# Autodesk Inventor assembly: PlattaAssembly
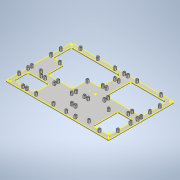
[picture p0: Inventor's stored thumbnail of the model, 180x180]
Saved by Autodesk Inventor 2021 (Build 250183000, 183)
## iProperties
Created: 2020-02-26
Part Number: PlattaAssembly
Document SubType Name: Assembly
Designer: lgnds
Author: lgnds
## Documents named in this file (3)
- C:\Users\Viktor\Documents\GitHub\WaveRunner-CCU\CCU_Assembly\hw\CAD\PlattaAssembly.iam
- C:\Users\Viktor\Documents\GitHub\WaveRunner-CCU\CCU_Assembly\hw\CAD\Platta.ipt
- C:\Users\Viktor\Documents\GitHub\WaveRunner-CCU\CCU_Assembly\hw\CAD\Other\Spacer7mm_m3_970070321.ipt
## Components (49 placed, 2 different names)
1. Platta:1 — Rigid:1, Rigid:2, Rigid:3, Rigid:4, Rigid:5, Rigid:6, Rigid:7, Rigid:8, Rigid:9, Rigid:10, Rigid:11, Rigid:12, Rigid:13, Rigid:14, Rigid:15, Rigid:16, Rigid:17, Rigid:18, Rigid:19, Rigid:20, Rigid:21, Rigid:22, Rigid:23, Rigid:24, Rigid:25, Rigid:26, Rigid:27, Rigid:28, Rigid:29, Rigid:30, Rigid:31, Rigid:32, Rigid:33, Rigid:34, Rigid:35, Rigid:36, Rigid:37, Rigid:38, Rigid:39, Rigid:40, Rigid:41, Rigid:42, Rigid:43, Rigid:44, Rigid:45, Rigid:46, Rigid:47, Rigid:48
2. Spacer7mm_m3_970070321:1 — Rigid:1
3. Spacer7mm_m3_970070321:2 — Rigid:2
4. Spacer7mm_m3_970070321:3 — Rigid:28
5. Spacer7mm_m3_970070321:4 — Rigid:29
6. Spacer7mm_m3_970070321:5 — Rigid:31
7. Spacer7mm_m3_970070321:6 — Rigid:33
8. Spacer7mm_m3_970070321:7 — Rigid:23
9. Spacer7mm_m3_970070321:8 — Rigid:24
10. Spacer7mm_m3_970070321:9 — Rigid:34
11. Spacer7mm_m3_970070321:10 — Rigid:47
12. Spacer7mm_m3_970070321:11 — Rigid:8
13. Spacer7mm_m3_970070321:12 — Rigid:7
14. Spacer7mm_m3_970070321:13 — Rigid:5
15. Spacer7mm_m3_970070321:14 — Rigid:4
16. Spacer7mm_m3_970070321:15 — Rigid:27
17. Spacer7mm_m3_970070321:16 — Rigid:26
18. Spacer7mm_m3_970070321:17 — Rigid:19
19. Spacer7mm_m3_970070321:18 — Rigid:17
20. Spacer7mm_m3_970070321:19 — Rigid:37
21. Spacer7mm_m3_970070321:20 — Rigid:14
22. Spacer7mm_m3_970070321:21 — Rigid:13
23. Spacer7mm_m3_970070321:22 — Rigid:12
24. Spacer7mm_m3_970070321:23 — Rigid:11
25. Spacer7mm_m3_970070321:24 — Rigid:25
26. Spacer7mm_m3_970070321:25 — Rigid:21
27. Spacer7mm_m3_970070321:26 — Rigid:18
28. Spacer7mm_m3_970070321:27 — Rigid:36
29. Spacer7mm_m3_970070321:28 — Rigid:16
30. Spacer7mm_m3_970070321:29 — Rigid:15
31. Spacer7mm_m3_970070321:30 — Rigid:38
32. Spacer7mm_m3_970070321:31 — Rigid:20
33. Spacer7mm_m3_970070321:32 — Rigid:22
34. Spacer7mm_m3_970070321:33 — Rigid:40
35. Spacer7mm_m3_970070321:34 — Rigid:41
36. Spacer7mm_m3_970070321:35 — Rigid:45
37. Spacer7mm_m3_970070321:36 — Rigid:46
38. Spacer7mm_m3_970070321:37 — Rigid:42
39. Spacer7mm_m3_970070321:38 — Rigid:39
40. Spacer7mm_m3_970070321:39 — Rigid:35
41. Spacer7mm_m3_970070321:40 — Rigid:32
42. Spacer7mm_m3_970070321:41 — Rigid:30
43. Spacer7mm_m3_970070321:42 — Rigid:44
44. Spacer7mm_m3_970070321:43 — Rigid:43
45. Spacer7mm_m3_970070321:44 — Rigid:3
46. Spacer7mm_m3_970070321:45 — Rigid:6
47. Spacer7mm_m3_970070321:46 — Rigid:48
48. Spacer7mm_m3_970070321:47 — Rigid:9
49. Spacer7mm_m3_970070321:48 — Rigid:10
## Relationships (48: WeldJoint 48)
- Rigid:1 [WeldJoint]: Platta:1 ↔ Spacer7mm_m3_970070321:1
- Rigid:2 [WeldJoint]: Platta:1 ↔ Spacer7mm_m3_970070321:2
- Rigid:3 [WeldJoint]: Platta:1 ↔ Spacer7mm_m3_970070321:44
- Rigid:4 [WeldJoint]: Platta:1 ↔ Spacer7mm_m3_970070321:14
- Rigid:5 [WeldJoint]: Platta:1 ↔ Spacer7mm_m3_970070321:13
- Rigid:6 [WeldJoint]: Platta:1 ↔ Spacer7mm_m3_970070321:45
- Rigid:7 [WeldJoint]: Platta:1 ↔ Spacer7mm_m3_970070321:12
- Rigid:8 [WeldJoint]: Platta:1 ↔ Spacer7mm_m3_970070321:11
- Rigid:9 [WeldJoint]: Platta:1 ↔ Spacer7mm_m3_970070321:47
- Rigid:10 [WeldJoint]: Platta:1 ↔ Spacer7mm_m3_970070321:48
- Rigid:11 [WeldJoint]: Platta:1 ↔ Spacer7mm_m3_970070321:23
- Rigid:12 [WeldJoint]: Platta:1 ↔ Spacer7mm_m3_970070321:22
- Rigid:13 [WeldJoint]: Platta:1 ↔ Spacer7mm_m3_970070321:21
- Rigid:14 [WeldJoint]: Platta:1 ↔ Spacer7mm_m3_970070321:20
- Rigid:15 [WeldJoint]: Platta:1 ↔ Spacer7mm_m3_970070321:29
- Rigid:16 [WeldJoint]: Platta:1 ↔ Spacer7mm_m3_970070321:28
- Rigid:17 [WeldJoint]: Platta:1 ↔ Spacer7mm_m3_970070321:18
- Rigid:18 [WeldJoint]: Platta:1 ↔ Spacer7mm_m3_970070321:26
- Rigid:19 [WeldJoint]: Platta:1 ↔ Spacer7mm_m3_970070321:17
- Rigid:20 [WeldJoint]: Platta:1 ↔ Spacer7mm_m3_970070321:31
- Rigid:21 [WeldJoint]: Platta:1 ↔ Spacer7mm_m3_970070321:25
- Rigid:22 [WeldJoint]: Platta:1 ↔ Spacer7mm_m3_970070321:32
- Rigid:23 [WeldJoint]: Platta:1 ↔ Spacer7mm_m3_970070321:7
- Rigid:24 [WeldJoint]: Platta:1 ↔ Spacer7mm_m3_970070321:8
- Rigid:25 [WeldJoint]: Platta:1 ↔ Spacer7mm_m3_970070321:24
- Rigid:26 [WeldJoint]: Platta:1 ↔ Spacer7mm_m3_970070321:16
- Rigid:27 [WeldJoint]: Platta:1 ↔ Spacer7mm_m3_970070321:15
- Rigid:28 [WeldJoint]: Platta:1 ↔ Spacer7mm_m3_970070321:3
- Rigid:29 [WeldJoint]: Platta:1 ↔ Spacer7mm_m3_970070321:4
- Rigid:30 [WeldJoint]: Platta:1 ↔ Spacer7mm_m3_970070321:41
- Rigid:31 [WeldJoint]: Platta:1 ↔ Spacer7mm_m3_970070321:5
- Rigid:32 [WeldJoint]: Platta:1 ↔ Spacer7mm_m3_970070321:40
- Rigid:33 [WeldJoint]: Platta:1 ↔ Spacer7mm_m3_970070321:6
- Rigid:34 [WeldJoint]: Platta:1 ↔ Spacer7mm_m3_970070321:9
- Rigid:35 [WeldJoint]: Platta:1 ↔ Spacer7mm_m3_970070321:39
- Rigid:36 [WeldJoint]: Platta:1 ↔ Spacer7mm_m3_970070321:27
- Rigid:37 [WeldJoint]: Platta:1 ↔ Spacer7mm_m3_970070321:19
- Rigid:38 [WeldJoint]: Platta:1 ↔ Spacer7mm_m3_970070321:30
- Rigid:39 [WeldJoint]: Platta:1 ↔ Spacer7mm_m3_970070321:38
- Rigid:40 [WeldJoint]: Platta:1 ↔ Spacer7mm_m3_970070321:33
- Rigid:41 [WeldJoint]: Platta:1 ↔ Spacer7mm_m3_970070321:34
- Rigid:42 [WeldJoint]: Platta:1 ↔ Spacer7mm_m3_970070321:37
- Rigid:43 [WeldJoint]: Platta:1 ↔ Spacer7mm_m3_970070321:43
- Rigid:44 [WeldJoint]: Platta:1 ↔ Spacer7mm_m3_970070321:42
- Rigid:45 [WeldJoint]: Platta:1 ↔ Spacer7mm_m3_970070321:35
- Rigid:46 [WeldJoint]: Platta:1 ↔ Spacer7mm_m3_970070321:36
- Rigid:47 [WeldJoint]: Platta:1 ↔ Spacer7mm_m3_970070321:10
- Rigid:48 [WeldJoint]: Platta:1 ↔ Spacer7mm_m3_970070321:46
